# Autodesk Inventor assembly: assembley
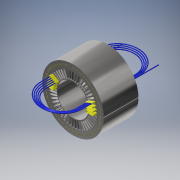
[picture p0: Inventor's stored thumbnail of the model, 180x180]
Saved by Autodesk Inventor 2018 (Build 220112000, 112)
## iProperties
Created: 2017-07-06
Part Number: assembley
Material: Типовые
Document SubType Name: Assembly
Designer: user
Author: user
## Documents named in this file (4)
- D:\WORK\MOLOT\WIRING_3\assembley.iam
- D:\WORK\MOLOT\WIRING_3\stator.ipt
- D:\WORK\MOLOT\WIRING_3\isolator_A.ipt
- D:\WORK\MOLOT\WIRING_3\winding_not_formed_A.ipt
## Components (50 placed, 3 different names)
1. stator:1 — Заподлицо:2, Совмещение:1, Совмещение:2, Совмещение:7, Заподлицо:4, Заподлицо:5
2. winding_not_formed_A:1 — Заподлицо:4, Заподлицо:5
3. isolator_A:1 — Заподлицо:3, Совмещение:3, Совмещение:4
4. isolator_A:2
5. isolator_A:3
6. isolator_A:4
7. isolator_A:49
8. isolator_A:6
9. isolator_A:7
10. isolator_A:8
11. isolator_A:9
12. isolator_A:10
13. isolator_A:11
14. isolator_A:12
15. isolator_A:13
16. isolator_A:14
17. isolator_A:15
18. isolator_A:16
19. isolator_A:17
20. isolator_A:18
21. isolator_A:19
22. isolator_A:20
23. isolator_A:21
24. isolator_A:22
25. isolator_A:23
26. isolator_A:24
27. isolator_A:25
28. isolator_A:26
29. isolator_A:27
30. isolator_A:28
31. isolator_A:29
32. isolator_A:30
33. isolator_A:31
34. isolator_A:32
35. isolator_A:33
36. isolator_A:34
37. isolator_A:35
38. isolator_A:36
39. isolator_A:37
40. isolator_A:38
41. isolator_A:39
42. isolator_A:40
43. isolator_A:41
44. isolator_A:42
45. isolator_A:43
46. isolator_A:44
47. isolator_A:45
48. isolator_A:46
49. isolator_A:47
50. isolator_A:48
## Component patterns: (48 elements, first: isolator_A:1)
## Relationships (11: Mate 7, Flush 4)
- Заподлицо:2 [Flush] (20 mm): stator:1
- Заподлицо:3 [Flush]: isolator_A:1
- Совмещение:1 [Mate]: stator:1
- Совмещение:2 [Mate]: stator:1
- Совмещение:3 [Mate]: isolator_A:1
- Совмещение:4 [Mate]: isolator_A:1
- Совмещение:5 [Mate]
- Совмещение:6 [Mate]
- Совмещение:7 [Mate]: stator:1
- Заподлицо:4 [Flush] (170 mm): stator:1 ↔ winding_not_formed_A:1
- Заподлицо:5 [Flush] (170 mm): stator:1 ↔ winding_not_formed_A:1
